# Autodesk Inventor assembly: Motor Assembly MH
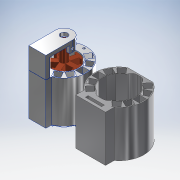
[picture p0: Inventor's stored thumbnail of the model, 180x180]
Saved by Autodesk Inventor 2018 (Build 220112000, 112)
## iProperties
Created: 2018-01-24
Part Number: Motor Assembly MH
Document SubType Name: Assembly
Designer: Moochster
Author: Moochster
## Documents named in this file (5)
- C:\Users\Moochster\OneDrive\Documents\2018 UBC\ELEC 391\Motor\SolidWorks\Motor Assembly MH.iam
- C:\Users\Moochster\OneDrive\Documents\2018 UBC\ELEC 391\Motor\SolidWorks\StatorShell MH.ipt
- C:\Users\Moochster\OneDrive\Documents\2018 UBC\ELEC 391\Motor\SolidWorks\RotorCore.ipt
- C:\Users\Moochster\OneDrive\Documents\2018 UBC\ELEC 391\Motor\SolidWorks\StatorShell.ipt
- C:\Users\Moochster\OneDrive\Documents\2018 UBC\ELEC 391\Motor\SolidWorks\Casing Attachment MH.ipt
## Components (4 placed, 4 different names)
1. StatorShell MH:1 — Mate:1, Flush:1, Mate:2, Flush:2
2. RotorCore:1 — Mate:1, Flush:1
3. StatorShell:1
4. Casing Attachment MH:1 — Mate:2, Flush:2
## Relationships (4: Mate 2, Flush 2)
- Mate:1: StatorShell MH:1 ↔ RotorCore:1
- Flush:1 (1 mm): StatorShell MH:1 ↔ RotorCore:1
- Mate:2: StatorShell MH:1 ↔ Casing Attachment MH:1
- Flush:2: StatorShell MH:1 ↔ Casing Attachment MH:1
